# Autodesk Inventor assembly: Panel asm
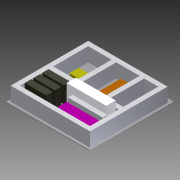
[picture p0: Inventor's stored thumbnail of the model, 180x180]
Saved by Autodesk Inventor 2014 (Build 180170000, 170)
## iProperties
Created: 2013-11-27
Part Number: Panel asm
Document SubType Name: Assembly
Designer: Devon
Author: Devon
## Documents named in this file (13)
- C:\Users\dclar4\Dropbox\ELEC 4497 - Senior Design\Design\Electrical\Panel asm.iam
- C:\Users\dclar4\Dropbox\ELEC 4497 - Senior Design\Design\Electrical\panel.ipt
- C:\Users\dclar4\Dropbox\ELEC 4497 - Senior Design\Design\Electrical\17in wire duct.ipt
- C:\Users\dclar4\Dropbox\ELEC 4497 - Senior Design\Design\Electrical\15in wire duct.ipt
- C:\Users\dclar4\Dropbox\ELEC 4497 - Senior Design\Design\Electrical\7.5in wire duct.ipt
- C:\Users\dclar4\Dropbox\ELEC 4497 - Senior Design\Design\Electrical\2x6.5 PCB.ipt
- C:\Users\dclar4\Dropbox\ELEC 4497 - Senior Design\Design\Electrical\Stepper Drive.ipt
- C:\Users\dclar4\Dropbox\ELEC 4497 - Senior Design\Design\Electrical\Power Suplply.ipt
- C:\Users\dclar4\Dropbox\ELEC 4497 - Senior Design\Design\Electrical\AND Gate.ipt
- C:\Users\dclar4\Dropbox\ELEC 4497 - Senior Design\Design\Electrical\chipkit.ipt
- C:\Users\dclar4\Dropbox\ELEC 4497 - Senior Design\Design\Electrical\IOIO.ipt
- C:\Users\dclar4\Dropbox\ELEC 4497 - Senior Design\Design\Electrical\relay board.ipt
- C:\Users\dclar4\Dropbox\ELEC 4497 - Senior Design\Design\Electrical\terminal block.ipt
## Components (19 placed, 12 different names)
1. panel:1 — Mate:1, Mate:2, Flush:1, Flush:2, Flush:3, Flush:4, Mate:3, Mate:4, Mate:5, Mate:15, Mate:19, Mate:22, Mate:26, Mate:27, Mate:28, Mate:37, Mate:38, Mate:39, Mate:40, Mate:41, Mate:53
2. 17in wire duct:1 — Mate:1, Flush:3, Flush:4, Mate:6, Flush:5, Mate:7, Flush:6, Mate:8, Mate:29, Mate:31, Mate:33, Mate:49, Mate:50
3. 17in wire duct:3 — Mate:2, Flush:1, Flush:2, Mate:24, Mate:35, Mate:55, Mate:57
4. 15in wire duct:1 — Mate:5, Mate:6, Flush:5, Mate:36, Mate:54
5. 15in wire duct:2 — Mate:4, Mate:8, Mate:30, Mate:44, Mate:51, Mate:58
6. 15in wire duct:3 — Mate:3, Mate:7, Flush:6, Mate:16, Mate:20, Mate:23, Mate:48
7. 7.5in wire duct:1 — Mate:15, Mate:16, Mate:42, Mate:43, Mate:47, Mate:52, Mate:58
8. 7.5in wire duct:2 — Mate:19, Mate:20
9. 2x6.5 PCB:1 — Mate:22, Mate:23, Mate:24
10. Stepper Drive:1 — Mate:26, Mate:31, Mate:32, Mate:34
11. Stepper Drive:2 — Mate:27, Mate:33, Mate:34
12. Stepper Drive:3 — Mate:28, Mate:29, Mate:30, Mate:32
13. Power Suplply:1 — Mate:35, Mate:36, Mate:37
14. AND Gate:1 — Mate:41, Mate:47, Mate:48
15. chipkit:1 — Mate:38, Mate:43, Mate:44, Mate:45, Mate:50
16. IOIO:1 — Mate:39, Mate:42, Mate:45, Mate:49
17. relay board:1 — Mate:40, Mate:51, Mate:52
18. terminal block:1 — Mate:53, Mate:54, Mate:55, Mate:56
19. 7.5in wire duct:3 — Mate:56, Mate:57
## Relationships (53: Mate 47, Flush 6)
- Mate:1: panel:1 ↔ 17in wire duct:1
- Mate:2: panel:1 ↔ 17in wire duct:3
- Flush:1 (12.7 mm): panel:1 ↔ 17in wire duct:3
- Flush:2 (12.7 mm): panel:1 ↔ 17in wire duct:3
- Flush:3 (12.7 mm): panel:1 ↔ 17in wire duct:1
- Flush:4 (12.7 mm): panel:1 ↔ 17in wire duct:1
- Mate:3: panel:1 ↔ 15in wire duct:3
- Mate:4: panel:1 ↔ 15in wire duct:2
- Mate:5: panel:1 ↔ 15in wire duct:1
- Mate:6: 17in wire duct:1 ↔ 15in wire duct:1
- Flush:5: 17in wire duct:1 ↔ 15in wire duct:1
- Mate:7: 17in wire duct:1 ↔ 15in wire duct:3
- Flush:6: 17in wire duct:1 ↔ 15in wire duct:3
- Mate:8: 17in wire duct:1 ↔ 15in wire duct:2
- Mate:15: panel:1 ↔ 7.5in wire duct:1
- Mate:16: 15in wire duct:3 ↔ 7.5in wire duct:1
- Mate:19: panel:1 ↔ 7.5in wire duct:2
- Mate:20: 15in wire duct:3 ↔ 7.5in wire duct:2
- Mate:22: panel:1 ↔ 2x6.5 PCB:1
- Mate:23 (12.7 mm): 15in wire duct:3 ↔ 2x6.5 PCB:1
- Mate:24 (12.7 mm): 17in wire duct:3 ↔ 2x6.5 PCB:1
- Mate:26: panel:1 ↔ Stepper Drive:1
- Mate:27: panel:1 ↔ Stepper Drive:2
- Mate:28: panel:1 ↔ Stepper Drive:3
- Mate:29 (12.7 mm): 17in wire duct:1 ↔ Stepper Drive:3
- Mate:30 (12.7 mm): 15in wire duct:2 ↔ Stepper Drive:3
- Mate:31 (12.7 mm): 17in wire duct:1 ↔ Stepper Drive:1
- Mate:32 (12.7 mm): Stepper Drive:1 ↔ Stepper Drive:3
- Mate:33 (12.7 mm): 17in wire duct:1 ↔ Stepper Drive:2
- Mate:34 (12.7 mm): Stepper Drive:1 ↔ Stepper Drive:2
- Mate:35 (12.7 mm): 17in wire duct:3 ↔ Power Suplply:1
- Mate:36 (101.6 mm): 15in wire duct:1 ↔ Power Suplply:1
- Mate:37: panel:1 ↔ Power Suplply:1
- Mate:38: panel:1 ↔ chipkit:1
- Mate:39: panel:1 ↔ IOIO:1
- Mate:40: panel:1 ↔ relay board:1
- Mate:41: panel:1 ↔ AND Gate:1
- Mate:42 (12.7 mm): 7.5in wire duct:1 ↔ IOIO:1
- Mate:43 (12.7 mm): 7.5in wire duct:1 ↔ chipkit:1
- Mate:44 (12.7 mm): 15in wire duct:2 ↔ chipkit:1
- Mate:45 (12.7 mm): chipkit:1 ↔ IOIO:1
- Mate:47 (25.4 mm): 7.5in wire duct:1 ↔ AND Gate:1
- Mate:48: 15in wire duct:3 ↔ AND Gate:1
- Mate:49 (12.7 mm): 17in wire duct:1 ↔ IOIO:1
- Mate:50 (12.7 mm): 17in wire duct:1 ↔ chipkit:1
- Mate:51 (6.35 mm): 15in wire duct:2 ↔ relay board:1
- Mate:52 (12.7 mm): 7.5in wire duct:1 ↔ relay board:1
- Mate:53: panel:1 ↔ terminal block:1
- Mate:54 (12.7 mm): 15in wire duct:1 ↔ terminal block:1
- Mate:55 (12.7 mm): 17in wire duct:3 ↔ terminal block:1
- Mate:56 (6.35 mm): terminal block:1 ↔ 7.5in wire duct:3
- Mate:57: 17in wire duct:3 ↔ 7.5in wire duct:3
- Mate:58: 15in wire duct:2 ↔ 7.5in wire duct:1
